# Autodesk Inventor assembly: SchaltkastenGesamt
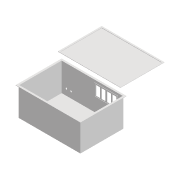
[picture p0: Inventor's stored thumbnail of the model, 180x180]
Saved by Autodesk Inventor 2021 (Build 250183000, 183)
## iProperties
Created: 2022-01-20
Part Number: SchaltkastenGesamt
Document SubType Name: Assembly
Designer: lukas
Author: lukas
## Documents named in this file (4)
- C:\Users\lukas\OneDrive - HTBLA Kaindorf\Diplomarbeit\Mechanik\InventorKonstruktion\SchaltkastenGesamt.iam
- C:\Users\lukas\OneDrive - HTBLA Kaindorf\Diplomarbeit\Mechanik\InventorKonstruktion\Deckel.ipt
- C:\Users\lukas\OneDrive - HTBLA Kaindorf\Diplomarbeit\Mechanik\InventorKonstruktion\Belüftung.ipt
- C:\Users\lukas\OneDrive - HTBLA Kaindorf\Diplomarbeit\Mechanik\InventorKonstruktion\Schaltkasten.ipt
## Components (3 placed, 3 different names)
1. Deckel:1
2. Belüftung:1 — Passend:1, Passend:2, Passend:3
3. Schaltkasten:1 — Passend:1, Passend:2, Passend:3
## Relationships (3: Mate 3)
- Passend:1 [Mate]: Belüftung:1 ↔ Schaltkasten:1
- Passend:2 [Mate]: Belüftung:1 ↔ Schaltkasten:1
- Passend:3 [Mate]: Belüftung:1 ↔ Schaltkasten:1
